# Autodesk Inventor assembly: HarmonicDrive
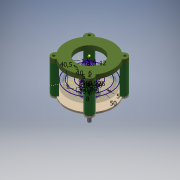
[picture p0: Inventor's stored thumbnail of the model, 180x180]
Saved by Autodesk Inventor 2018.3 (Build 223284000, 284)
## iProperties
Created: 2018-06-22
Part Number: HarmonicDrive
Material: Generisch
Document SubType Name: Assembly
Designer: JochenAlt
Author: JochenAlt
## Documents named in this file (8)
- D:\Projects\FlowerPot\CAD\HarmonicDrive.iam
- D:\Projects\FlowerPot\CAD\HarmonicDrive.ipt
- D:\Projects\FlowerPot\CAD\CircularSpline.ipt
- C:\Users\JochenAlt\Documents\Inventor\Content Center Files\R2018\de-DE\SKF - Single row ball bearings\SKF604.ipt
- D:\Projects\FlowerPot\CAD\HarmonicDrive-WaveGenerator-Bottom.ipt
- D:\Projects\FlowerPot\CAD\Mounting Hub.ipt
- D:\Projects\FlowerPot\CAD\HarmonicDrive-Axis.ipt
- C:\Users\JochenAlt\Documents\Inventor\Content Center Files\R2018\de-DE\AS 1420\AS 1420 - 1973 - M3 x 6.ipt
## Components (12 placed, 7 different names)
1. Harmonic Drive:1 — Passend:12, Passend:13, Passend:17, Passend:19, Passend:22
2. CircularSpline:1 — Passend:12, Passend:13, Passend:14, Passend:20, Passend:21, Einfügen:1, Einfügen:2, Einfügen:3, Einfügen:4
3. SKF- Kugellager, einreihig SKF604:2 — Passend:9, Passend:14, Passend:15
4. SKF- Kugellager, einreihig SKF604:1 — Passend:7, Passend:16
5. HarmonicDrive-WaveGenerator-Bottom:1 — Passend:7, Passend:9, Passend:15, Passend:16, Passend:17
6. Mounting Hub:1 — Passend:18, Passend:19, Passend:20, Passend:21, Passend:23, Fluchtend:1, Passend:24
7. HarmonicDrive-Axis:1 — Passend:18, Fluchtend:1, Passend:25
8. AS 1420 - Metrisch M3 x 6:1 — Einfügen:1
9. AS 1420 - Metrisch M3 x 6:2 — Einfügen:2, Passend:24
10. AS 1420 - Metrisch M3 x 6:3 — Einfügen:3
11. AS 1420 - Metrisch M3 x 6:4 — Einfügen:4
12. SKF- Kugellager, einreihig SKF604:3 — Passend:22, Passend:23, Passend:25
## Relationships (21: Mate 16, Insert 4, Flush 1)
- Passend:7 [Mate] (0.5 mm): SKF- Kugellager, einreihig SKF604:1 ↔ HarmonicDrive-WaveGenerator-Bottom:1
- Passend:9 [Mate] (0.5 mm): SKF- Kugellager, einreihig SKF604:2 ↔ HarmonicDrive-WaveGenerator-Bottom:1
- Passend:12 [Mate] (25 mm): Harmonic Drive:1 ↔ CircularSpline:1
- Passend:13 [Mate]: Harmonic Drive:1 ↔ CircularSpline:1
- Passend:14 [Mate]: CircularSpline:1 ↔ SKF- Kugellager, einreihig SKF604:2
- Passend:15 [Mate]: SKF- Kugellager, einreihig SKF604:2 ↔ HarmonicDrive-WaveGenerator-Bottom:1
- Passend:16 [Mate]: SKF- Kugellager, einreihig SKF604:1 ↔ HarmonicDrive-WaveGenerator-Bottom:1
- Passend:17 [Mate]: Harmonic Drive:1 ↔ HarmonicDrive-WaveGenerator-Bottom:1
- Passend:18 [Mate]: Mounting Hub:1 ↔ HarmonicDrive-Axis:1
- Passend:19 [Mate]: Harmonic Drive:1 ↔ Mounting Hub:1
- Passend:20 [Mate]: CircularSpline:1 ↔ Mounting Hub:1
- Passend:21 [Mate]: CircularSpline:1 ↔ Mounting Hub:1
- Einfügen:1 [Insert]: CircularSpline:1 ↔ AS 1420 - Metrisch M3 x 6:1
- Einfügen:2 [Insert]: CircularSpline:1 ↔ AS 1420 - Metrisch M3 x 6:2
- Einfügen:3 [Insert]: CircularSpline:1 ↔ AS 1420 - Metrisch M3 x 6:3
- Einfügen:4 [Insert]: CircularSpline:1 ↔ AS 1420 - Metrisch M3 x 6:4
- Passend:22 [Mate]: Harmonic Drive:1 ↔ SKF- Kugellager, einreihig SKF604:3
- Passend:23 [Mate]: Mounting Hub:1 ↔ SKF- Kugellager, einreihig SKF604:3
- Fluchtend:1 [Flush]: Mounting Hub:1 ↔ HarmonicDrive-Axis:1
- Passend:24 [Mate]: Mounting Hub:1 ↔ AS 1420 - Metrisch M3 x 6:2
- Passend:25 [Mate]: HarmonicDrive-Axis:1 ↔ SKF- Kugellager, einreihig SKF604:3
